# Autodesk Inventor assembly: base mg996r 3mm frame
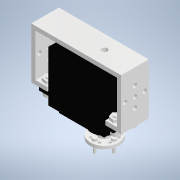
[picture p0: Inventor's stored thumbnail of the model, 180x180]
Saved by Autodesk Inventor 2021.4 (Build 254397000, 397)
## iProperties
Created: 2022-07-09
Part Number: base mg996r 3mm frame
Document SubType Name: Assembly
Designer: isamu
Author: isamu
## Documents named in this file (7)
- D:\personal_projects\robot\inventor\2021\base mg996r 3mm frame.iam
- D:\personal_projects\robot\exports\servo motors\servo-motor-mg996r servo.ipt
- D:\personal_projects\robot\exports\frames\servo frame.ipt
- D:\personal_projects\robot\exports\handle\servo handle 4.ipt
- D:\personal_projects\robot\exports\screws\m4x8.ipt
- D:\personal_projects\robot\exports\screws\m4 nuts.ipt
- D:\personal_projects\robot\exports\screws\m2x8.ipt
## Components (15 placed, 6 different names)
1. servo-motor-mg996r servo:1 — Mate:1, Mate:2, Mate:3, Insert:1, Insert:2, Insert:3, Insert:4, Rotational:1
2. servo frame:1 — Mate:1, Mate:2, Mate:3, Insert:5, Insert:6, Insert:7, Insert:8
3. m4x8:1 — Insert:1
4. m4x8:2 — Insert:2
5. m4x8:3 — Insert:4
6. m4x8:4 — Insert:3
7. m4 nuts:1 — Insert:8
8. m4 nuts:2 — Insert:7
9. m4 nuts:3 — Insert:5
10. m4 nuts:4 — Insert:6
11. m2x8:1 — Insert:12
12. m2x8:2 — Insert:11
13. m2x8:3 — Insert:9
14. m2x8:4 — Insert:10
15. servo handle 4:1 — Rotational:1, Insert:9, Insert:10, Insert:11, Insert:12
## Relationships (16: Insert 12, Mate 3, RevoluteJoint 1)
- Mate:1: servo-motor-mg996r servo:1 ↔ servo frame:1
- Mate:2: servo-motor-mg996r servo:1 ↔ servo frame:1
- Mate:3: servo-motor-mg996r servo:1 ↔ servo frame:1
- Insert:1: servo-motor-mg996r servo:1 ↔ m4x8:1
- Insert:2: servo-motor-mg996r servo:1 ↔ m4x8:2
- Insert:3: servo-motor-mg996r servo:1 ↔ m4x8:4
- Insert:4: servo-motor-mg996r servo:1 ↔ m4x8:3
- Insert:5: servo frame:1 ↔ m4 nuts:3
- Insert:6: servo frame:1 ↔ m4 nuts:4
- Insert:7: servo frame:1 ↔ m4 nuts:2
- Insert:8: servo frame:1 ↔ m4 nuts:1
- Rotational:1 [RevoluteJoint]: servo-motor-mg996r servo:1 ↔ servo handle 4:1
- Insert:9: m2x8:3 ↔ servo handle 4:1
- Insert:10: m2x8:4 ↔ servo handle 4:1
- Insert:11: m2x8:2 ↔ servo handle 4:1
- Insert:12: m2x8:1 ↔ servo handle 4:1
